# Autodesk Inventor assembly: 3.25 Omni AS, No Insert
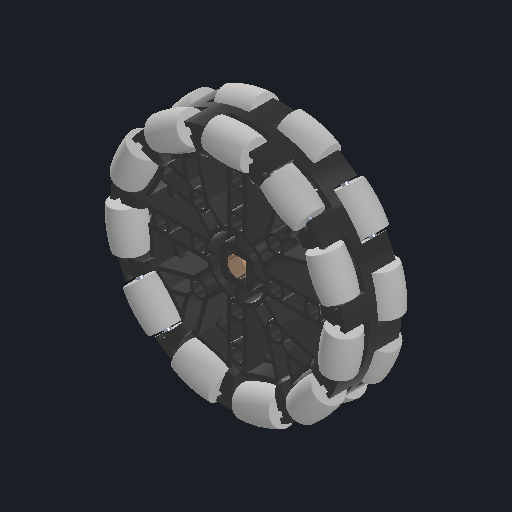
[picture p0: Inventor's stored thumbnail of the model, 512x512]
Saved by Autodesk Inventor 2025 (Build 290162000, 162)
## iProperties
Created: 2022-08-02
Part Number: 3.25 Omni AS, No Insert
Document SubType Name: Assembly
Designer: Averey Ku
Author: ylu12
## Documents named in this file (2)
- D:\VEX\High Stakes\CAD\V5\Chassis\Drivebay Right\3.25 Omni AS, No Insert.iam
- D:\VEX\High Stakes\CAD\V5\Chassis\Drivebay Right\3.25 Omni Antistatic.ipt
## Components (1 placed, 1 different names)
1. 3.25 Omni Antistatic:1 — Mate:12, Mate:11, Flush:6
## Relationships (3: Mate 2, Flush 1)
- Mate:12: 3.25 Omni Antistatic:1
- Mate:11: 3.25 Omni Antistatic:1
- Flush:6: 3.25 Omni Antistatic:1
